# Autodesk Inventor assembly: ModeloBase
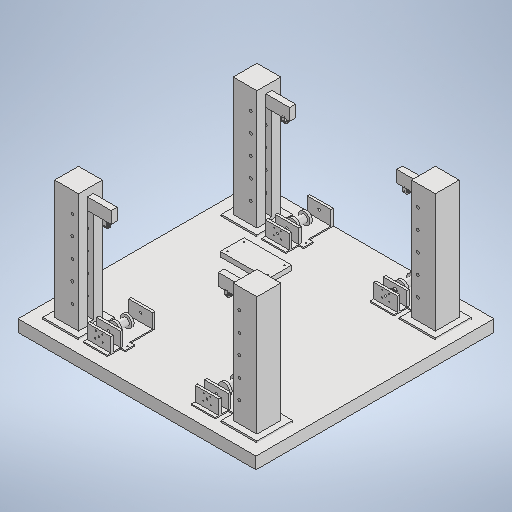
[picture p0: Inventor's stored thumbnail of the model, 512x512]
Saved by Autodesk Inventor 2026 (Build 300175050, 175E)
## iProperties
Created: 2025-04-13
Part Number: ModeloBase
Document SubType Name: Assembly
Designer: piero
Author: piero
## Documents named in this file (12)
- C:\Users\piero\OneDrive\Documentos\UTEC\Ciclo 2025-1\PFC_1\ModeloBase\ModeloBase.iam
- C:\Users\piero\OneDrive\Documentos\UTEC\Ciclo 2025-1\PFC_1\ModeloBase\Base.ipt
- C:\Users\piero\OneDrive\Documentos\UTEC\Ciclo 2025-1\PFC_1\ModeloBase\Plataforma.ipt
- C:\Users\piero\OneDrive\Documentos\UTEC\Ciclo 2025-1\PFC_1\ModeloBase\Torres.ipt
- C:\Users\piero\OneDrive\Documentos\UTEC\Ciclo 2025-1\PFC_1\ModeloBase\polea.ipt
- C:\Users\piero\OneDrive\Documentos\Inventor\Content Center Files\R2024\es-ES\JIS B 1189\JIS B 1189 - M14 x 2 - 110.ipt
- C:\Users\piero\OneDrive\Documentos\Inventor\Content Center Files\R2024\es-ES\JIS B 1182(1)\JIS B 1182 - M4x25.ipt
- C:\Users\piero\OneDrive\Documentos\UTEC\Ciclo 2025-1\PFC_1\ModeloBase\BaseMotor.ipt
- C:\Users\piero\OneDrive\Documentos\UTEC\Ciclo 2025-1\PFC_1\ModeloBase\nema17\17HM15-0904S.iam
- C:\Users\piero\OneDrive\Documentos\UTEC\Ciclo 2025-1\PFC_1\ModeloBase\Base_motor.ipt
- C:\Users\piero\OneDrive\Documentos\UTEC\Ciclo 2025-1\PFC_1\ModeloBase\carrete.ipt
- C:\Users\piero\OneDrive\Documentos\UTEC\Ciclo 2025-1\PFC_1\ModeloBase\acople_suave.ipt
## Components (29 placed, 11 different names)
1. Base:2 — Nivelación:3, Nivelación:5, Nivelación:6, Nivelación:7
2. Plataforma:1 — Nivelación:3, Nivelación:5
3. Torres:1 — Coincidencia:4, Coincidencia:5, Coincidencia:6, Coincidencia:7, Coincidencia:8, Insertar:1, Insertar:2, Insertar:3
4. polea:4 — Coincidencia:4, Insertar:8
5. polea:8 — Coincidencia:6, Insertar:6
6. polea:9 — Coincidencia:5, Insertar:7
7. polea:10 — Coincidencia:7, Insertar:9
8. JIS B 1189 - Métrico M14 x 110:1 — Coincidencia:8
9. JIS B 1189 - Métrico M14 x 110:2 — Insertar:1
10. JIS B 1189 - Métrico M14 x 110:3 — Insertar:2
11. JIS B 1189 - Métrico M14 x 110:4 — Insertar:3
12. JIS B 1182 Final achaflanado - Métrico M4x25:1 — Insertar:6
13. JIS B 1182 Final achaflanado - Métrico M4x25:2 — Insertar:7
14. JIS B 1182 Final achaflanado - Métrico M4x25:3 — Insertar:8
15. JIS B 1182 Final achaflanado - Métrico M4x25:4 — Insertar:9
16. BaseMotor:1 — Nivelación:6, Nivelación:7, Coincidencia:12, Coincidencia:13, Coincidencia:14, Coincidencia:15
17. 17HM15-0904S:3 [sub-assembly] — Coincidencia:15
18. 17HM15-0904S:6 [sub-assembly] — Coincidencia:14
19. 17HM15-0904S:7 [sub-assembly] — Coincidencia:13
20. 17HM15-0904S:8 [sub-assembly] — Coincidencia:12
21. Base_motor:1
22. Base_motor:2
23. Base_motor:3
24. Base_motor:4
25. carrete:1
26. carrete:2
27. carrete:3
28. carrete:4
29. acople_suave:3
## Relationships (20: Mate 9, Insert 7, Flush 4)
- Nivelación:3 [Flush]: Base:2 ↔ Plataforma:1
- Nivelación:5 [Flush] (-500 mm): Base:2 ↔ Plataforma:1
- Coincidencia:4 [Mate]: Torres:1 ↔ polea:4
- Coincidencia:5 [Mate]: Torres:1 ↔ polea:9
- Coincidencia:6 [Mate]: Torres:1 ↔ polea:8
- Coincidencia:7 [Mate]: Torres:1 ↔ polea:10
- Coincidencia:8 [Mate]: Torres:1 ↔ JIS B 1189 - Métrico M14 x 110:1
- Insertar:1: Torres:1 ↔ JIS B 1189 - Métrico M14 x 110:2
- Insertar:2: Torres:1 ↔ JIS B 1189 - Métrico M14 x 110:3
- Insertar:3: Torres:1 ↔ JIS B 1189 - Métrico M14 x 110:4
- Insertar:6: polea:8 ↔ JIS B 1182 Final achaflanado - Métrico M4x25:1
- Insertar:7: polea:9 ↔ JIS B 1182 Final achaflanado - Métrico M4x25:2
- Insertar:8: polea:4 ↔ JIS B 1182 Final achaflanado - Métrico M4x25:3
- Insertar:9: polea:10 ↔ JIS B 1182 Final achaflanado - Métrico M4x25:4
- Nivelación:6 [Flush]: Base:2 ↔ BaseMotor:1
- Nivelación:7 [Flush]: Base:2 ↔ BaseMotor:1
- Coincidencia:12 [Mate]: BaseMotor:1 ↔ 17HM15-0904S:8
- Coincidencia:13 [Mate]: BaseMotor:1 ↔ 17HM15-0904S:7
- Coincidencia:14 [Mate]: BaseMotor:1 ↔ 17HM15-0904S:6
- Coincidencia:15 [Mate]: BaseMotor:1 ↔ 17HM15-0904S:3
